# Autodesk Inventor assembly: Scale
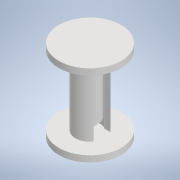
[picture p0: Inventor's stored thumbnail of the model, 180x180]
Saved by Autodesk Inventor 2022 (Build 260153000, 153)
## iProperties
Created: 2021-10-23
Part Number: Scale
Document SubType Name: Assembly
Designer: liwei
Author: liwei
## Documents named in this file (3)
- D:\Documents\HackGT\HackGT8-Food-Analyzer\Scale.iam
- D:\Documents\HackGT\HackGT8-Food-Analyzer\fsrBase.ipt
- D:\Documents\HackGT\HackGT8-Food-Analyzer\fsrTop.ipt
## Components (2 placed, 2 different names)
1. fsrBase:1 — Cylindrical:1
2. fsrTop:1 — Cylindrical:1
## Relationships (1: CylindricalJoint 1)
- Cylindrical:1: fsrBase:1 ↔ fsrTop:1
